# Autodesk Inventor assembly: MMBOT
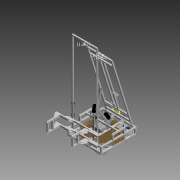
[picture p0: Inventor's stored thumbnail of the model, 180x180]
Saved by Autodesk Inventor 2013 (Build 170138000, 138)
## iProperties
Created: 2015-01-07
Part Number: MMBOT
Document SubType Name: Assembly
Designer: darkb_000
Mass: 41457 g
Surface Area: 57368.6 cm^2
Volume: 21063.5 cm^3
Density: 1.96819 g/cm^3
Author: darkb_000
## Documents named in this file (38)
- C:\Users\eedoga.OHSD\Desktop\proswishper011115\2015-Robot-master\Swish\MMBOT.iam
- C:\Users\eedoga.OHSD\Desktop\proswishper011115\2015-Robot-master\Swish\BotLayoutGLass.ipt
- C:\Users\eedoga.OHSD\Desktop\proswishper011115\2015-Robot-master\Swish\Cchannel27inch.ipt
- C:\Users\eedoga.OHSD\Desktop\proswishper011115\2015-Robot-master\Swish\Chassis_Channel_26_AndyMark_am-0202.ipt
- C:\Users\eedoga.OHSD\Desktop\proswishper011115\2015-Robot-master\Swish\Chassis_CornerConnect_AndyMark_am-0212.ipt
- C:\Users\eedoga.OHSD\Desktop\proswishper011115\2015-Robot-master\Swish\HolonomicCornerBracket.ipt
- C:\Users\eedoga.OHSD\Desktop\proswishper011115\2015-Robot-master\Swish\HolonomicCornerBracket02.ipt
- C:\Users\eedoga.OHSD\Desktop\proswishper011115\2015-Robot-master\Swish\Toughbox-nano-500-key-long-asm.iam
- C:\Users\eedoga.OHSD\Desktop\proswishper011115\2015-Robot-master\Swish\8-Molded-Trick-Wheel.iam
- C:\Users\eedoga.OHSD\Desktop\proswishper011115\2015-Robot-master\Swish\HolonomicCornerBracket_MIR.ipt
- C:\Users\eedoga.OHSD\Desktop\proswishper011115\2015-Robot-master\Swish\HolonomicCornerBracket02_MIR.ipt
- C:\Users\eedoga.OHSD\Desktop\proswishper011115\2015-Robot-master\Swish\Toughbox-nano-500-key-long-asm_MIR.iam
- C:\Users\eedoga.OHSD\Desktop\proswishper011115\2015-Robot-master\Swish\8-Molded-Trick-Wheel_MIR.iam
- C:\Users\eedoga.OHSD\Desktop\proswishper011115\2015-Robot-master\Swish\HolonomicCornerBracket_MIR1.ipt
- C:\Users\eedoga.OHSD\Desktop\proswishper011115\2015-Robot-master\Swish\HolonomicCornerBracket02_MIR1.ipt
- C:\Users\eedoga.OHSD\Desktop\proswishper011115\2015-Robot-master\Swish\Toughbox-nano-500-key-long-asm_MIR1.iam
- C:\Users\eedoga.OHSD\Desktop\proswishper011115\2015-Robot-master\Swish\8-Molded-Trick-Wheel_MIR1.iam
- C:\Users\eedoga.OHSD\Desktop\proswishper011115\2015-Robot-master\Swish\HolonomicCornerBracket_MIR_MIR.ipt
- C:\Users\eedoga.OHSD\Desktop\proswishper011115\2015-Robot-master\Swish\HolonomicCornerBracket02_MIR_MIR.ipt
- C:\Users\eedoga.OHSD\Desktop\proswishper011115\2015-Robot-master\Swish\Toughbox-nano-500-key-long-asm_MIR_MIR.iam
- C:\Users\eedoga.OHSD\Desktop\proswishper011115\2015-Robot-master\Swish\8-Molded-Trick-Wheel_MIR_MIR.iam
- C:\Users\eedoga.OHSD\Desktop\proswishper011115\2015-Robot-master\Swish\3inchUp.ipt
- C:\Users\eedoga.OHSD\Desktop\proswishper011115\2015-Robot-master\Swish\SideLong.ipt
- C:\Users\eedoga.OHSD\Desktop\proswishper011115\2015-Robot-master\Swish\backlong.ipt
- C:\Users\eedoga.OHSD\Desktop\proswishper011115\2015-Robot-master\Swish\channelBracket02.ipt
- C:\Users\eedoga.OHSD\Desktop\proswishper011115\2015-Robot-master\Swish\8020-1010 54upthingy.ipt
- C:\Users\eedoga.OHSD\Desktop\proswishper011115\2015-Robot-master\Swish\6715.iam
- C:\Users\eedoga.OHSD\Desktop\proswishper011115\2015-Robot-master\Swish\MMMainLiftTopCrossBar.ipt
- C:\Users\eedoga.OHSD\Desktop\proswishper011115\2015-Robot-master\Swish\mmCenterTowerCross01.ipt
- C:\Users\eedoga.OHSD\Desktop\CAD Files\Imported Components\DARTActuator12\DARTActuator12.iam
- C:\Users\eedoga.OHSD\Desktop\proswishper011115\2015-Robot-master\Swish\batassj115.iam
- C:\Users\eedoga.OHSD\Desktop\Electronics Base.ipt
- C:\Users\eedoga.OHSD\Desktop\Battery mechanism motor assembly.iam
- C:\Users\eedoga.OHSD\Desktop\RandallLiftMech\RandalLiftMech.iam
- C:\Users\eedoga.OHSD\Desktop\proswishper011115\2015-Robot-master\Swish\armmount01.ipt
- C:\Users\eedoga.OHSD\Desktop\RandallLiftMech\PullySystemSmall.iam
- C:\Users\eedoga.OHSD\Desktop\proswishper011115\2015-Robot-master\Swish\dartmount.ipt
- C:\Users\eedoga.OHSD\Desktop\proswishper011115\2015-Robot-master\Swish\Gripper\gripperAss.iam
## Components (63 placed, 37 different names)
1. BotLayoutGLass:1 — Flush:1, Flush:2, Flush:4, Mate:19
2. Cchannel27inch:1 — Flush:1, Flush:2, Flush:5, Mate:1, Mate:2, Mate:5, Mate:7, Mate:8, Flush:7, Mate:19, Flush:10, Flush:11
3. Cchannel27inch:2 — Flush:4, Flush:5, Mate:13, Mate:14, Mate:15, Mate:16, Flush:51
4. Chassis_Channel_26_AndyMark_am-0202:1 — Mate:9, Mate:10, Flush:7, Mate:17, Mate:18
5. Chassis_Channel_26_AndyMark_am-0202:2 — Mate:3, Mate:4, Mate:6, Mate:11, Mate:12, Flush:50
6. Chassis_CornerConnect_AndyMark_am-0212:1 — Mate:11, Mate:12, Mate:13, Mate:14, Flush:8, Flush:9
7. Chassis_CornerConnect_AndyMark_am-0212:2 — Mate:15, Mate:16, Mate:17, Mate:18, Flush:9
8. Chassis_CornerConnect_AndyMark_am-0212:3 — Mate:7, Mate:8, Mate:9, Mate:10, Flush:6
9. Chassis_CornerConnect_AndyMark_am-0212:4 — Mate:1, Mate:2, Mate:3, Mate:4, Mate:5, Mate:6, Flush:6, Flush:8
10. HolonomicCornerBracket:1 — Flush:10, Mate:23, Mate:36, Flush:17, Flush:18
11. HolonomicCornerBracket02:1 — Flush:11, Mate:20, Mate:21, Flush:12
12. Toughbox-nano-500-key-long-asm:1 [sub-assembly] — Mate:20, Mate:21, Flush:12, Mate:22
13. 8-Molded-Trick-Wheel:1 [sub-assembly] — Mate:22, Mate:23
14. HolonomicCornerBracket_MIR:1 — Mate:26, Flush:16
15. HolonomicCornerBracket02_MIR:1 — Flush:13, Mate:24, Mate:25
16. Toughbox-nano-500-key-long-asm_MIR:1 [sub-assembly] — Flush:13, Mate:24, Mate:25, Mate:27
17. 8-Molded-Trick-Wheel_MIR:1 [sub-assembly] — Mate:26, Mate:27
18. HolonomicCornerBracket_MIR1:1 — Mate:30, Mate:37, Flush:19, Flush:20
19. HolonomicCornerBracket02_MIR1:1 — Flush:14, Mate:28, Mate:29, Mate:75
20. Toughbox-nano-500-key-long-asm_MIR1:1 [sub-assembly] — Flush:14, Mate:28, Mate:29, Mate:31
21. 8-Molded-Trick-Wheel_MIR1:1 [sub-assembly] — Mate:30, Mate:31
22. HolonomicCornerBracket_MIR_MIR:1 — Mate:35, Mate:38, Flush:21, Flush:22
23. HolonomicCornerBracket02_MIR_MIR:1 — Mate:32, Mate:33, Flush:15
24. Toughbox-nano-500-key-long-asm_MIR_MIR:1 [sub-assembly] — Mate:32, Mate:33, Flush:15, Mate:34
25. 8-Molded-Trick-Wheel_MIR_MIR:1 [sub-assembly] — Mate:34, Mate:35
26. 3inchUp:1 — Flush:16, Flush:27
27. 3inchUp:2 — Mate:36, Flush:17, Flush:18, Flush:24, Flush:25, Mate:39
28. 3inchUp:3 — Mate:37, Flush:19, Flush:20
29. 3inchUp:4 — Mate:38, Flush:21, Flush:22, Flush:23
30. SideLong:1 — Flush:23, Flush:26, Mate:40, Flush:28, Mate:68, Flush:41, Mate:69, Flush:42
31. SideLong:2 — Flush:24, Flush:25, Mate:39, Flush:31, Mate:65, Flush:39, Mate:66, Flush:40, Flush:45
32. backlong:1 — Flush:26, Mate:76, Mate:77, Mate:78, Mate:79, Mate:80, Mate:81, Mate:82, Mate:83
33. backlong:2 — Mate:40, Flush:27, Flush:28, Mate:41, Mate:42, Mate:43, Mate:44, Flush:32, Mate:72, Mate:73, Mate:74
34. channelBracket02:1 — Mate:43, Mate:44, Mate:49, Mate:52, Mate:53, Flush:52, Flush:54
35. channelBracket02:2 — Mate:41, Mate:42, Mate:49, Flush:31, Mate:50, Mate:51, Mate:63, Flush:53
36. 8020-1010 54upthingy:1 — Mate:50, Mate:51, Flush:32, Flush:33, Mate:54, Mate:55, Mate:58, Mate:59, Flush:38, Mate:64
37. 8020-1010 54upthingy:2 — Mate:52, Mate:53, Flush:33, Mate:56, Mate:57, Mate:60, Mate:61
38. 6715:1 [sub-assembly] — Mate:54, Mate:55, Flush:34, Flush:35
39. 6715:2 [sub-assembly] — Mate:56, Mate:57, Flush:34, Flush:35, Mate:118
40. 6715:3 [sub-assembly] — Mate:58, Mate:59, Flush:36, Flush:37, Flush:58, Mate:111, Mate:112, Mate:113, Flush:59
41. 6715:4 [sub-assembly] — Mate:60, Mate:61, Flush:36, Flush:37, Flush:58, Mate:116, Flush:59, Mate:117, Mate:118
42. MMMainLiftTopCrossBar:1 — Mate:63, Flush:38, Mate:64, Mate:98, Mate:99, Mate:100
43. DARTActuator12:1 [sub-assembly] — Mate:104, Mate:105
44. DARTActuator12:2 [sub-assembly] — Mate:109, Mate:110
45. 3inchUp:5 — Mate:69, Flush:42, Flush:43
46. 3inchUp:6 — Mate:68, Flush:41, Flush:44, Mate:71, Flush:48, Flush:49
47. 3inchUp:7 — Mate:66, Flush:40, Mate:67, Flush:44, Flush:45, Mate:70, Flush:46, Flush:47
48. 3inchUp:8 — Mate:65, Flush:39, Mate:67, Flush:43
49. mmCenterTowerCross01:1 — Mate:70, Flush:46, Flush:47
50. mmCenterTowerCross01:2 — Mate:71, Flush:48, Flush:49, Mate:86, Flush:56, Flush:57
51. batassj115:1 [sub-assembly] — Mate:72, Mate:73, Mate:74
52. Electronics Base:1 — Mate:75, Flush:50, Flush:51
53. Battery mechanism motor assembly:1 [sub-assembly] — Mate:76, Mate:77, Mate:78, Mate:79
54. RandalLiftMech:1 [sub-assembly] — Mate:84, Mate:85
55. channelBracket02:3 — Mate:80, Mate:81, Flush:52, Flush:54, Mate:84, Mate:85
56. channelBracket02:4 — Mate:82, Mate:83, Flush:53
57. backlong:3 — Mate:86, Flush:56, Flush:57, Mate:101, Mate:102, Mate:103, Mate:106, Mate:107, Mate:108
58. PullySystemSmall:1 [sub-assembly] — Mate:98, Mate:99, Mate:100
59. dartmount:1 — Mate:101, Mate:102, Mate:103, Mate:104, Mate:105
60. dartmount:2 — Mate:106, Mate:107, Mate:108, Mate:109, Mate:110
61. armmount01:1 — Mate:111, Mate:112, Mate:113, Flush:60, Flush:61, Flush:62, Mate:119, Mate:120
62. armmount01:2 — Mate:116, Flush:60, Mate:117
63. gripperAss:1 [sub-assembly] — Flush:61, Flush:62, Mate:119, Mate:120
## Relationships (160: Mate 102, Flush 58)
- Flush:1: BotLayoutGLass:1 ↔ Cchannel27inch:1
- Flush:2: BotLayoutGLass:1 ↔ Cchannel27inch:1
- Flush:4: BotLayoutGLass:1 ↔ Cchannel27inch:2
- Flush:5: Cchannel27inch:1 ↔ Cchannel27inch:2
- Mate:1: Cchannel27inch:1 ↔ Chassis_CornerConnect_AndyMark_am-0212:4
- Mate:2: Cchannel27inch:1 ↔ Chassis_CornerConnect_AndyMark_am-0212:4
- Mate:3: Chassis_Channel_26_AndyMark_am-0202:2 ↔ Chassis_CornerConnect_AndyMark_am-0212:4
- Mate:4: Chassis_Channel_26_AndyMark_am-0202:2 ↔ Chassis_CornerConnect_AndyMark_am-0212:4
- Mate:5: Cchannel27inch:1 ↔ Chassis_CornerConnect_AndyMark_am-0212:4
- Mate:6: Chassis_Channel_26_AndyMark_am-0202:2 ↔ Chassis_CornerConnect_AndyMark_am-0212:4
- Mate:7: Cchannel27inch:1 ↔ Chassis_CornerConnect_AndyMark_am-0212:3
- Mate:8: Cchannel27inch:1 ↔ Chassis_CornerConnect_AndyMark_am-0212:3
- Mate:9: Chassis_Channel_26_AndyMark_am-0202:1 ↔ Chassis_CornerConnect_AndyMark_am-0212:3
- Mate:10: Chassis_Channel_26_AndyMark_am-0202:1 ↔ Chassis_CornerConnect_AndyMark_am-0212:3
- Flush:6: Chassis_CornerConnect_AndyMark_am-0212:3 ↔ Chassis_CornerConnect_AndyMark_am-0212:4
- Flush:7: Cchannel27inch:1 ↔ Chassis_Channel_26_AndyMark_am-0202:1
- Mate:11: Chassis_Channel_26_AndyMark_am-0202:2 ↔ Chassis_CornerConnect_AndyMark_am-0212:1
- Mate:12: Chassis_Channel_26_AndyMark_am-0202:2 ↔ Chassis_CornerConnect_AndyMark_am-0212:1
- Mate:13: Cchannel27inch:2 ↔ Chassis_CornerConnect_AndyMark_am-0212:1
- Mate:14: Cchannel27inch:2 ↔ Chassis_CornerConnect_AndyMark_am-0212:1
- Flush:8: Chassis_CornerConnect_AndyMark_am-0212:1 ↔ Chassis_CornerConnect_AndyMark_am-0212:4
- Mate:15: Cchannel27inch:2 ↔ Chassis_CornerConnect_AndyMark_am-0212:2
- Mate:16: Cchannel27inch:2 ↔ Chassis_CornerConnect_AndyMark_am-0212:2
- Mate:17: Chassis_Channel_26_AndyMark_am-0202:1 ↔ Chassis_CornerConnect_AndyMark_am-0212:2
- Mate:18: Chassis_Channel_26_AndyMark_am-0202:1 ↔ Chassis_CornerConnect_AndyMark_am-0212:2
- Flush:9: Chassis_CornerConnect_AndyMark_am-0212:1 ↔ Chassis_CornerConnect_AndyMark_am-0212:2
- Mate:19 (101.6 mm): BotLayoutGLass:1 ↔ Cchannel27inch:1
- Flush:10: Cchannel27inch:1 ↔ HolonomicCornerBracket:1
- Flush:11: Cchannel27inch:1 ↔ HolonomicCornerBracket02:1
- Mate:20: HolonomicCornerBracket02:1 ↔ Toughbox-nano-500-key-long-asm:1
- Mate:21: HolonomicCornerBracket02:1 ↔ Toughbox-nano-500-key-long-asm:1
- Flush:12: HolonomicCornerBracket02:1 ↔ Toughbox-nano-500-key-long-asm:1
- Mate:22: Toughbox-nano-500-key-long-asm:1 ↔ 8-Molded-Trick-Wheel:1
- Mate:23 (25.4 mm): HolonomicCornerBracket:1 ↔ 8-Molded-Trick-Wheel:1
- Flush:13: HolonomicCornerBracket02_MIR:1 ↔ Toughbox-nano-500-key-long-asm_MIR:1
- Mate:24: HolonomicCornerBracket02_MIR:1 ↔ Toughbox-nano-500-key-long-asm_MIR:1
- Mate:25: HolonomicCornerBracket02_MIR:1 ↔ Toughbox-nano-500-key-long-asm_MIR:1
- Mate:26 (25.4 mm): HolonomicCornerBracket_MIR:1 ↔ 8-Molded-Trick-Wheel_MIR:1
- Mate:27: Toughbox-nano-500-key-long-asm_MIR:1 ↔ 8-Molded-Trick-Wheel_MIR:1
- Flush:14: HolonomicCornerBracket02_MIR1:1 ↔ Toughbox-nano-500-key-long-asm_MIR1:1
- Mate:28: HolonomicCornerBracket02_MIR1:1 ↔ Toughbox-nano-500-key-long-asm_MIR1:1
- Mate:29: HolonomicCornerBracket02_MIR1:1 ↔ Toughbox-nano-500-key-long-asm_MIR1:1
- Mate:30 (25.4 mm): HolonomicCornerBracket_MIR1:1 ↔ 8-Molded-Trick-Wheel_MIR1:1
- Mate:31: Toughbox-nano-500-key-long-asm_MIR1:1 ↔ 8-Molded-Trick-Wheel_MIR1:1
- Mate:32: HolonomicCornerBracket02_MIR_MIR:1 ↔ Toughbox-nano-500-key-long-asm_MIR_MIR:1
- Mate:33: HolonomicCornerBracket02_MIR_MIR:1 ↔ Toughbox-nano-500-key-long-asm_MIR_MIR:1
- Flush:15: HolonomicCornerBracket02_MIR_MIR:1 ↔ Toughbox-nano-500-key-long-asm_MIR_MIR:1
- Mate:34: Toughbox-nano-500-key-long-asm_MIR_MIR:1 ↔ 8-Molded-Trick-Wheel_MIR_MIR:1
- Mate:35 (25.4 mm): HolonomicCornerBracket_MIR_MIR:1 ↔ 8-Molded-Trick-Wheel_MIR_MIR:1
- Flush:16: HolonomicCornerBracket_MIR:1 ↔ 3inchUp:1
- Mate:36: HolonomicCornerBracket:1 ↔ 3inchUp:2
- Flush:17: HolonomicCornerBracket:1 ↔ 3inchUp:2
- Flush:18: HolonomicCornerBracket:1 ↔ 3inchUp:2
- Mate:37: HolonomicCornerBracket_MIR1:1 ↔ 3inchUp:3
- Flush:19: HolonomicCornerBracket_MIR1:1 ↔ 3inchUp:3
- Flush:20: HolonomicCornerBracket_MIR1:1 ↔ 3inchUp:3
- Mate:38: HolonomicCornerBracket_MIR_MIR:1 ↔ 3inchUp:4
- Flush:21: HolonomicCornerBracket_MIR_MIR:1 ↔ 3inchUp:4
- Flush:22: HolonomicCornerBracket_MIR_MIR:1 ↔ 3inchUp:4
- Flush:23: 3inchUp:4 ↔ SideLong:1
- Flush:24: 3inchUp:2 ↔ SideLong:2
- Flush:25: 3inchUp:2 ↔ SideLong:2
- Mate:39: 3inchUp:2 ↔ SideLong:2
- Flush:26: SideLong:1 ↔ backlong:1
- Mate:40: SideLong:1 ↔ backlong:2
- Flush:27: 3inchUp:1 ↔ backlong:2
- Flush:28: SideLong:1 ↔ backlong:2
- Mate:41: backlong:2 ↔ channelBracket02:2
- Mate:42: backlong:2 ↔ channelBracket02:2
- Mate:43: backlong:2 ↔ channelBracket02:1
- Mate:44: backlong:2 ↔ channelBracket02:1
- Mate:49 (457.2 mm): channelBracket02:1 ↔ channelBracket02:2
- Flush:31 (-82.55 mm): SideLong:2 ↔ channelBracket02:2
- Mate:50: channelBracket02:2 ↔ 8020-1010 54upthingy:1
- Mate:51: channelBracket02:2 ↔ 8020-1010 54upthingy:1
- Flush:32: backlong:2 ↔ 8020-1010 54upthingy:1
- Mate:52: channelBracket02:1 ↔ 8020-1010 54upthingy:2
- Mate:53: channelBracket02:1 ↔ 8020-1010 54upthingy:2
- Flush:33: 8020-1010 54upthingy:1 ↔ 8020-1010 54upthingy:2
- Mate:54: 8020-1010 54upthingy:1 ↔ 6715:1
- Mate:55: 8020-1010 54upthingy:1 ↔ 6715:1
- Mate:56: 8020-1010 54upthingy:2 ↔ 6715:2
- Mate:57: 8020-1010 54upthingy:2 ↔ 6715:2
- Flush:34: 6715:1 ↔ 6715:2
- Flush:35: 6715:1 ↔ 6715:2
- Mate:58: 8020-1010 54upthingy:1 ↔ 6715:3
- Mate:59: 8020-1010 54upthingy:1 ↔ 6715:3
- Mate:60: 8020-1010 54upthingy:2 ↔ 6715:4
- Mate:61: 8020-1010 54upthingy:2 ↔ 6715:4
- Flush:36: 6715:3 ↔ 6715:4
- Flush:37: 6715:3 ↔ 6715:4
- Mate:63: channelBracket02:2 ↔ MMMainLiftTopCrossBar:1
- Flush:38: 8020-1010 54upthingy:1 ↔ MMMainLiftTopCrossBar:1
- Mate:64: 8020-1010 54upthingy:1 ↔ MMMainLiftTopCrossBar:1
- Mate:65: SideLong:2 ↔ 3inchUp:8
- Flush:39: SideLong:2 ↔ 3inchUp:8
- Mate:66: SideLong:2 ↔ 3inchUp:7
- Flush:40: SideLong:2 ↔ 3inchUp:7
- Mate:67 (203.2 mm): 3inchUp:7 ↔ 3inchUp:8
- Mate:68: SideLong:1 ↔ 3inchUp:6
- Flush:41: SideLong:1 ↔ 3inchUp:6
- Mate:69: SideLong:1 ↔ 3inchUp:5
- Flush:42: SideLong:1 ↔ 3inchUp:5
- Flush:43: 3inchUp:5 ↔ 3inchUp:8
- Flush:44: 3inchUp:6 ↔ 3inchUp:7
- Flush:45 (228.6 mm): SideLong:2 ↔ 3inchUp:7
- Mate:70: 3inchUp:7 ↔ mmCenterTowerCross01:1
- Flush:46: 3inchUp:7 ↔ mmCenterTowerCross01:1
- Flush:47: 3inchUp:7 ↔ mmCenterTowerCross01:1
- Mate:71: 3inchUp:6 ↔ mmCenterTowerCross01:2
- Flush:48: 3inchUp:6 ↔ mmCenterTowerCross01:2
- Flush:49: 3inchUp:6 ↔ mmCenterTowerCross01:2
- Mate:72: backlong:2 ↔ batassj115:1
- Mate:73: backlong:2 ↔ batassj115:1
- Mate:74: backlong:2 ↔ batassj115:1
- Mate:75: HolonomicCornerBracket02_MIR1:1 ↔ Electronics Base:1
- Flush:50: Chassis_Channel_26_AndyMark_am-0202:2 ↔ Electronics Base:1
- Flush:51: Cchannel27inch:2 ↔ Electronics Base:1
- Mate:76: backlong:1 ↔ Battery mechanism motor assembly:1
- Mate:77: backlong:1 ↔ Battery mechanism motor assembly:1
- Mate:78: backlong:1 ↔ Battery mechanism motor assembly:1
- Mate:79: backlong:1 ↔ Battery mechanism motor assembly:1
- Mate:80: backlong:1 ↔ channelBracket02:3
- Mate:81: backlong:1 ↔ channelBracket02:3
- Flush:52: channelBracket02:1 ↔ channelBracket02:3
- Mate:82: backlong:1 ↔ channelBracket02:4
- Mate:83: backlong:1 ↔ channelBracket02:4
- Flush:53: channelBracket02:2 ↔ channelBracket02:4
- Flush:54: channelBracket02:1 ↔ channelBracket02:3
- Mate:84: RandalLiftMech:1 ↔ channelBracket02:3
- Mate:85: RandalLiftMech:1 ↔ channelBracket02:3
- Mate:86: mmCenterTowerCross01:2 ↔ backlong:3
- Flush:56: mmCenterTowerCross01:2 ↔ backlong:3
- Flush:57 (114.3 mm): mmCenterTowerCross01:2 ↔ backlong:3
- Mate:98: MMMainLiftTopCrossBar:1 ↔ PullySystemSmall:1
- Mate:99: MMMainLiftTopCrossBar:1 ↔ PullySystemSmall:1
- Mate:100: MMMainLiftTopCrossBar:1 ↔ PullySystemSmall:1
- Mate:101: backlong:3 ↔ dartmount:1
- Mate:102: backlong:3 ↔ dartmount:1
- Mate:103: backlong:3 ↔ dartmount:1
- Mate:104: DARTActuator12:1 ↔ dartmount:1
- Mate:105 (12.7 mm): DARTActuator12:1 ↔ dartmount:1
- Mate:106: backlong:3 ↔ dartmount:2
- Mate:107: backlong:3 ↔ dartmount:2
- Mate:108: backlong:3 ↔ dartmount:2
- Mate:109: DARTActuator12:2 ↔ dartmount:2
- Mate:110 (12.7 mm): DARTActuator12:2 ↔ dartmount:2
- Flush:58: 6715:3 ↔ 6715:4
- Mate:111: 6715:3 ↔ armmount01:1
- Mate:112: 6715:3 ↔ armmount01:1
- Mate:113: 6715:3 ↔ armmount01:1
- Mate:116: 6715:4 ↔ armmount01:2
- Flush:59: 6715:3 ↔ 6715:4
- Flush:60: armmount01:1 ↔ armmount01:2
- Mate:117: 6715:4 ↔ armmount01:2
- Mate:118 (-254 mm): 6715:2 ↔ 6715:4
- Flush:61: armmount01:1 ↔ gripperAss:1
- Flush:62: armmount01:1 ↔ gripperAss:1
- Mate:119: armmount01:1 ↔ gripperAss:1
- Mate:120: armmount01:1 ↔ gripperAss:1
